# Autodesk Inventor assembly: !drivebay_mirrored
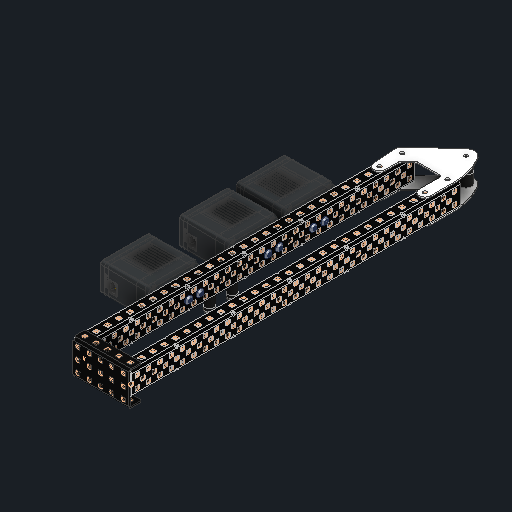
[picture p0: Inventor's stored thumbnail of the model, 512x512]
Saved by Autodesk Inventor 2024 (Build 280153000, 153)
## iProperties
Created: 2024-05-13
Part Number: !drivebay_mirrored
Document SubType Name: Assembly
Designer: Averey Ku
Author: Averey Ku
## Documents named in this file (13)
- D:\vex_robotics\hardware\cad\kdot\chassis\drivebay\mirrored_parts\!drivebay_mirrored.iam
- D:\vex_robotics\hardware\cad\kdot\chassis\drivebay\mirrored_parts\outer_mirrored.iam
- D:\vex_robotics\hardware\cad\kdot\chassis\drivebay\mirrored_parts\inner_mirrored.iam
- D:\vex_robotics\hardware\cad\kdot\chassis\drivebay\mirrored_parts\Alu C 1x2x1x5_mirrored.ipt
- D:\vex_robotics\hardware\cad\kdot\chassis\drivebay\mirrored_parts\gusset_mirrored.ipt
- D:\vex_robotics\hardware\cad\VEX-CAD-Inventor-1.41\Motion\Spacers\Spacer Nylon .500 OD\NSpacer Black .500 OD x .500.ipt
- D:\vex_robotics\hardware\cad\VEX-CAD-Inventor-1.41\Motion\Spacers\Spacer Nylon .500 OD.ipt
- D:\vex_robotics\hardware\cad\kdot\chassis\drivebay\mirrored_parts\Alu C 1x3x1x5_mirrored.ipt
- D:\vex_robotics\hardware\cad\VEX-CAD-Inventor-1.41\Motion\Spacers\Spacer Nylon .375 OD\NSpacer .375 OD x .125.ipt
- D:\vex_robotics\hardware\cad\VEX-CAD-Inventor-1.41\Motion\Spacers\Spacer Nylon .375 OD.ipt
- D:\vex_robotics\hardware\cad\VEX-CAD-Inventor-1.41\Motion\Spacers\Spacer Nylon .375 OD\NSpacer .375 OD x .500.ipt
- D:\vex_robotics\hardware\cad\VEX-CAD-Inventor-1.41\Motion\Spacers\Washer Steel\SWasher .375 OD x .062500.ipt
- D:\vex_robotics\hardware\cad\VEX-CAD-Inventor-1.41\Motion\Spacers\Washer Steel.ipt
## Components (14 placed, 9 different names)
1. outer_mirrored:1 [sub-assembly] — Mate:1, Insert:1, Mate:4, Insert:4, Mate:6
2. inner_mirrored:1 [sub-assembly] — Mate:2, Insert:2, Mate:3, Insert:3, Mate:5, Insert:5, Insert:8, Insert:11, Insert:12
3. Alu C 1x2x1x5_mirrored:1 — Mate:2, Insert:2, Mate:1, Insert:1
4. gusset_mirrored:1 — Mate:4, Insert:4, Mate:3, Insert:3, Insert:7
5. gusset_mirrored:2 — Mate:5, Insert:5
6. NSpacer Black .500 OD x .500:1 — Insert:6
7. NSpacer Black .500 OD x .500:2 — Insert:7, Insert:6
8. Alu C 1x3x1x5_mirrored:1 — Mate:6, Insert:8
9. NSpacer .375 OD x .125:1 — Insert:9, Insert:14
10. NSpacer .375 OD x .500:2 — Insert:11, Insert:9
11. NSpacer .375 OD x .125:3 — Insert:10, Insert:13
12. NSpacer .375 OD x .500:4 — Insert:12, Insert:10
13. SWasher .375 OD x .062500:1 — Insert:14
14. SWasher .375 OD x .062500:2 — Insert:13
## Relationships (20: Insert 14, Mate 6)
- Mate:2: inner_mirrored:1 ↔ Alu C 1x2x1x5_mirrored:1
- Insert:2: inner_mirrored:1 ↔ Alu C 1x2x1x5_mirrored:1
- Mate:1: outer_mirrored:1 ↔ Alu C 1x2x1x5_mirrored:1
- Insert:1: outer_mirrored:1 ↔ Alu C 1x2x1x5_mirrored:1
- Mate:4: outer_mirrored:1 ↔ gusset_mirrored:1
- Insert:4: outer_mirrored:1 ↔ gusset_mirrored:1
- Mate:3: inner_mirrored:1 ↔ gusset_mirrored:1
- Insert:3: inner_mirrored:1 ↔ gusset_mirrored:1
- Mate:5: inner_mirrored:1 ↔ gusset_mirrored:2
- Insert:5: inner_mirrored:1 ↔ gusset_mirrored:2
- Insert:7: gusset_mirrored:1 ↔ NSpacer Black .500 OD x .500:2
- Insert:6: NSpacer Black .500 OD x .500:1 ↔ NSpacer Black .500 OD x .500:2
- Mate:6: outer_mirrored:1 ↔ Alu C 1x3x1x5_mirrored:1
- Insert:8: inner_mirrored:1 ↔ Alu C 1x3x1x5_mirrored:1
- Insert:11: inner_mirrored:1 ↔ NSpacer .375 OD x .500:2
- Insert:9: NSpacer .375 OD x .125:1 ↔ NSpacer .375 OD x .500:2
- Insert:12: inner_mirrored:1 ↔ NSpacer .375 OD x .500:4
- Insert:10: NSpacer .375 OD x .125:3 ↔ NSpacer .375 OD x .500:4
- Insert:14: NSpacer .375 OD x .125:1 ↔ SWasher .375 OD x .062500:1
- Insert:13: NSpacer .375 OD x .125:3 ↔ SWasher .375 OD x .062500:2
